# Autodesk Inventor assembly: Ensamblaje1
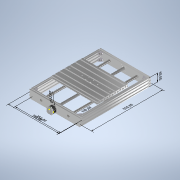
[picture p0: Inventor's stored thumbnail of the model, 180x180]
Saved by Autodesk Inventor 2021 (Build 250183000, 183)
## iProperties
Created: 2022-05-21
Part Number: Ensamblaje1
Document SubType Name: Assembly
Designer: 79449
Author: 79449
## Documents named in this file (27)
- C:\Users\79449\Documents\CNC_DISENO_DE MAQUINAS\Piezas-Ensambles_Inventor\Primera_presentación\Ensamblaje1.iam
- C:\Users\79449\Documents\CNC_DISENO_DE MAQUINAS\Piezas-Ensambles_Inventor\Primera_presentación\V-SLOT_2060_26cm.ipt
- C:\Users\79449\Documents\CNC_DISENO_DE MAQUINAS\Piezas-Ensambles_Inventor\Primera_presentación\V-SLOT_2060_30cm.ipt
- C:\Users\79449\Documents\CNC_DISENO_DE MAQUINAS\Piezas-Ensambles_Inventor\Primera_presentación\SFU-1605.ipt
- C:\Users\79449\Documents\CNC_DISENO_DE MAQUINAS\Piezas-Ensambles_Inventor\Primera_presentación\Ball Screew.step.ipt
- C:\Users\79449\Documents\CNC_DISENO_DE MAQUINAS\Piezas-Ensambles_Inventor\Primera_presentación\EjeBase.ipt
- C:\Users\79449\Documents\CNC_DISENO_DE MAQUINAS\Piezas-Ensambles_Inventor\Primera_presentación\ball nut housing bracket holder.ipt
- C:\Users\79449\Documents\CNC_DISENO_DE MAQUINAS\Piezas-Ensambles_Inventor\Primera_presentación\Chumacera\chumacera de 20 mm.iam
- C:\Users\79449\Documents\CNC_DISENO_DE MAQUINAS\Piezas-Ensambles_Inventor\Primera_presentación\T_20240.ipt
- C:\Users\79449\Documents\Inventor\Content Center Files\R2021\es-ES\AS 1427(05)\AS 1427 - M8 x 30(5) II.ipt
- C:\Users\79449\Documents\CNC_DISENO_DE MAQUINAS\Piezas-Ensambles_Inventor\Primera_presentación\PiezaNivel.ipt
- C:\Users\79449\Documents\Inventor\Content Center Files\R2021\es-ES\AS 1427(05)\AS 1427 - M4 x 20(5) II.ipt
- C:\Users\79449\Documents\CNC_DISENO_DE MAQUINAS\Piezas-Ensambles_Inventor\Primera_presentación\Cast corner bracket-20x20x17.ipt
- C:\Users\79449\Documents\Inventor\Content Center Files\R2021\es-ES\ANSI_ASME B18.5\ANSI_ASME B18.5 - 1_4 - 20 - 7_16 - 1_4-20 UNC.ipt
- C:\Users\79449\Documents\CNC_DISENO_DE MAQUINAS\Piezas-Ensambles_Inventor\Primera_presentación\Cast corner bracket-20x20x17_MIR.ipt
- C:\Users\79449\Documents\CNC_DISENO_DE MAQUINAS\Piezas-Ensambles_Inventor\Primera_presentación\Cast corner bracket-20x20x17_MIR1.ipt
- C:\Users\79449\Documents\CNC_DISENO_DE MAQUINAS\Piezas-Ensambles_Inventor\Primera_presentación\Cast corner bracket-20x20x17_MIR_MIR.ipt
- C:\Users\79449\Documents\Inventor\Content Center Files\R2021\es-ES\ANSI B18.2.2(08)\ANSI B18.2.2 - 1_4 - 20(3).ipt
- C:\Users\79449\Documents\Inventor\Content Center Files\R2021\es-ES\SAE J773b\SAE J773b - 3_8. SAE Tipo L. Fino.ipt
- C:\Users\79449\Documents\Inventor\Content Center Files\R2021\es-ES\AS 1112 (2)\AS 1112 - M8  Tipo 10.ipt
- C:\Users\79449\Documents\CNC_DISENO_DE MAQUINAS\Piezas-Ensambles_Inventor\Primera_presentación\Cast corner bracket-20x20x17_MIR2.ipt
- C:\Users\79449\Documents\CNC_DISENO_DE MAQUINAS\Piezas-Ensambles_Inventor\Primera_presentación\Cast corner bracket-20x20x17_MIR_MIR1.ipt
- C:\Users\79449\Documents\CNC_DISENO_DE MAQUINAS\Piezas-Ensambles_Inventor\Primera_presentación\Cast corner bracket-20x20x17_MIR1_MIR.ipt
- C:\Users\79449\Documents\CNC_DISENO_DE MAQUINAS\Piezas-Ensambles_Inventor\Primera_presentación\Cast corner bracket-20x20x17_MIR_MIR_MIR.ipt
- C:\Users\79449\Documents\CNC_DISENO_DE MAQUINAS\Piezas-Ensambles_Inventor\Primera_presentación\Nema17\Assembly1.iam
- C:\Users\79449\Documents\CNC_DISENO_DE MAQUINAS\Piezas-Ensambles_Inventor\Primera_presentación\Flexible Coupling 16-5.ipt
- C:\Users\79449\Documents\Inventor\Content Center Files\R2021\es-ES\U 3284(2)\Unbrako. Hallowell Steel Collars. Inch Series - 0.625 x 1 1_8 x 1_2.ipt
## Components (72 placed, 27 different names)
1. V-SLOT_2060_51cm:1 — Coincidencia:1, Coincidencia:3, Coincidencia:4, Coincidencia:6, Coincidencia:10, Coincidencia:11, Coincidencia:12, Coincidencia:52, Coincidencia:63
2. V-SLOT_2060_30cm:1 — Coincidencia:8, Coincidencia:10, Coincidencia:12, Coincidencia:14, Coincidencia:17, Coincidencia:19, Coincidencia:53, Coincidencia:60, Simetría:1
3. V-SLOT_2060_51cm:2 — Coincidencia:2, Coincidencia:3, Coincidencia:13
4. V-SLOT_2060_39cm:2 — Coincidencia:4, Coincidencia:5, Coincidencia:6, Coincidencia:13, Coincidencia:18, Coincidencia:20, Nivelación:3, Simetría:1, Ángulo:2, Coincidencia:124, Coincidencia:125, Coincidencia:131
5. SFU-1605:1 — Coincidencia:16, Coincidencia:21, Nivelación:1, Coincidencia:22
6. Ball Screew.step:1 — Coincidencia:14, Coincidencia:16, Coincidencia:126, Coincidencia:129
7. EjeBase:1 — Coincidencia:17, Coincidencia:18, Coincidencia:24
8. EjeBase:2 — Coincidencia:19, Coincidencia:20, Coincidencia:23, Coincidencia:130
9. ball nut housing bracket holder:1 — Coincidencia:21, Nivelación:1, Coincidencia:22, Ángulo:1, Coincidencia:38, Coincidencia:39
10. chumacera de 20 mm:1 [sub-assembly] — Coincidencia:23, Coincidencia:25, Coincidencia:35, Coincidencia:87, Coincidencia:89
11. chumacera de 20 mm:2 [sub-assembly] — Coincidencia:24, Coincidencia:26, Coincidencia:29, Coincidencia:31, Coincidencia:91, Coincidencia:93
12. T_20240:1 — Coincidencia:25, Coincidencia:26, Coincidencia:27, Coincidencia:28, Coincidencia:30, Coincidencia:32, Coincidencia:33, Coincidencia:34, Coincidencia:35, Coincidencia:36, Coincidencia:37, Ángulo:1, Coincidencia:41, Coincidencia:43, Coincidencia:45, Coincidencia:46, Coincidencia:47, Coincidencia:48, Coincidencia:49, Coincidencia:50
13. AS 1427 H - Métrico M8 x 30:1 — Coincidencia:34, Coincidencia:37, Coincidencia:88, Coincidencia:100
14. AS 1427 H - Métrico M8 x 30:3 — Coincidencia:33, Coincidencia:36, Coincidencia:86, Coincidencia:98
15. AS 1427 H - Métrico M8 x 30:4 — Coincidencia:27, Coincidencia:28, Coincidencia:29, Coincidencia:92, Coincidencia:94
16. AS 1427 H - Métrico M8 x 30:7 — Coincidencia:30, Coincidencia:31, Coincidencia:32, Coincidencia:90, Coincidencia:96
17. PiezaNivel:1 — Coincidencia:38, Coincidencia:39, Coincidencia:51
18. AS 1427 H - Métrico M4 x 20:1 — Coincidencia:41, Coincidencia:49
19. AS 1427 H - Métrico M4 x 20:2 — Coincidencia:43, Coincidencia:46
20. AS 1427 H - Métrico M4 x 20:3 — Coincidencia:45, Coincidencia:50
21. AS 1427 H - Métrico M4 x 20:5 — Coincidencia:47, Coincidencia:48, Coincidencia:51
22. Cast corner bracket-20x20x17:2 — Coincidencia:52, Coincidencia:53, Coincidencia:61, Coincidencia:62, Coincidencia:64, Coincidencia:71, Coincidencia:73
23. Perno de cabeza en T - Pulgadas 1/4 - 20 - 7/16:1 — Coincidencia:60, Coincidencia:61, Coincidencia:72
24. Perno de cabeza en T - Pulgadas 1/4 - 20 - 7/16:2 — Coincidencia:62, Coincidencia:63, Coincidencia:70
25. Cast corner bracket-20x20x17_MIR:1 — Coincidencia:65, Coincidencia:75, Coincidencia:77
26. Perno de cabeza en T - Pulgadas 1/4 - 20 - 7/16:3 — Coincidencia:76
27. Perno de cabeza en T - Pulgadas 1/4 - 20 - 7/16:4 — Coincidencia:74
28. Cast corner bracket-20x20x17_MIR1:1 — Coincidencia:66, Coincidencia:83, Coincidencia:85
29. Perno de cabeza en T - Pulgadas 1/4 - 20 - 7/16:5 — Coincidencia:84
30. Perno de cabeza en T - Pulgadas 1/4 - 20 - 7/16:6 — Coincidencia:82
31. Cast corner bracket-20x20x17_MIR_MIR:1 — Coincidencia:69, Coincidencia:79, Coincidencia:81
32. Perno de cabeza en T - Pulgadas 1/4 - 20 - 7/16:7 — Coincidencia:78
33. Perno de cabeza en T - Pulgadas 1/4 - 20 - 7/16:8 — Coincidencia:80
34. Tuerca de apriete hex - Pulgadas 1/4 - 20:1 — Coincidencia:70, Coincidencia:71
35. Tuerca de apriete hex - Pulgadas 1/4 - 20:2 — Coincidencia:72, Coincidencia:73
36. Tuerca de apriete hex - Pulgadas 1/4 - 20:3 — Coincidencia:74, Coincidencia:75
37. Tuerca de apriete hex - Pulgadas 1/4 - 20:4 — Coincidencia:76, Coincidencia:77
38. Tuerca de apriete hex - Pulgadas 1/4 - 20:5 — Coincidencia:78, Coincidencia:79
39. Tuerca de apriete hex - Pulgadas 1/4 - 20:6 — Coincidencia:80, Coincidencia:81
40. Tuerca de apriete hex - Pulgadas 1/4 - 20:7 — Coincidencia:82, Coincidencia:83
41. Tuerca de apriete hex - Pulgadas 1/4 - 20:8 — Coincidencia:84, Coincidencia:85
42. Arandela elástica SAE J773b (Pulgadas) 3/8. SAE Tipo L. Fino:1 — Coincidencia:86, Coincidencia:87, Coincidencia:99
43. Arandela elástica SAE J773b (Pulgadas) 3/8. SAE Tipo L. Fino:2 — Coincidencia:88, Coincidencia:89, Coincidencia:101
44. Arandela elástica SAE J773b (Pulgadas) 3/8. SAE Tipo L. Fino:3 — Coincidencia:90, Coincidencia:91, Coincidencia:97
45. Arandela elástica SAE J773b (Pulgadas) 3/8. SAE Tipo L. Fino:4 — Coincidencia:92, Coincidencia:93, Coincidencia:95
46. AS 1112 (2) - Métrico M8  Tipo 10:1 — Coincidencia:94, Coincidencia:95
47. AS 1112 (2) - Métrico M8  Tipo 10:2 — Coincidencia:96, Coincidencia:97
48. AS 1112 (2) - Métrico M8  Tipo 10:3 — Coincidencia:98, Coincidencia:99
49. AS 1112 (2) - Métrico M8  Tipo 10:4 — Coincidencia:100, Coincidencia:101
50. Cast corner bracket-20x20x17_MIR2:1 — Coincidencia:102, Coincidencia:108, Coincidencia:110
51. Perno de cabeza en T - Pulgadas 1/4 - 20 - 7/16:9 — Coincidencia:111
52. Perno de cabeza en T - Pulgadas 1/4 - 20 - 7/16:10 — Coincidencia:109
53. Cast corner bracket-20x20x17_MIR_MIR1:1 — Coincidencia:105, Coincidencia:112, Coincidencia:114
54. Perno de cabeza en T - Pulgadas 1/4 - 20 - 7/16:11 — Coincidencia:115
55. Perno de cabeza en T - Pulgadas 1/4 - 20 - 7/16:12 — Coincidencia:113
56. Cast corner bracket-20x20x17_MIR1_MIR:1 — Coincidencia:106, Coincidencia:120, Coincidencia:122
57. Perno de cabeza en T - Pulgadas 1/4 - 20 - 7/16:13 — Coincidencia:123
58. Perno de cabeza en T - Pulgadas 1/4 - 20 - 7/16:14 — Coincidencia:121
59. Cast corner bracket-20x20x17_MIR_MIR_MIR:1 — Coincidencia:107, Coincidencia:116, Coincidencia:118
60. Perno de cabeza en T - Pulgadas 1/4 - 20 - 7/16:15 — Coincidencia:117
61. Perno de cabeza en T - Pulgadas 1/4 - 20 - 7/16:16 — Coincidencia:119
62. Tuerca de apriete hex - Pulgadas 1/4 - 20:9 — Coincidencia:108, Coincidencia:109
63. Tuerca de apriete hex - Pulgadas 1/4 - 20:10 — Coincidencia:110, Coincidencia:111
64. Tuerca de apriete hex - Pulgadas 1/4 - 20:11 — Coincidencia:112, Coincidencia:113
65. Tuerca de apriete hex - Pulgadas 1/4 - 20:12 — Coincidencia:114, Coincidencia:115
66. Tuerca de apriete hex - Pulgadas 1/4 - 20:13 — Coincidencia:116, Coincidencia:117
67. Tuerca de apriete hex - Pulgadas 1/4 - 20:14 — Coincidencia:118, Coincidencia:119
68. Tuerca de apriete hex - Pulgadas 1/4 - 20:15 — Coincidencia:120, Coincidencia:121
69. Tuerca de apriete hex - Pulgadas 1/4 - 20:16 — Coincidencia:122, Coincidencia:123
70. Assembly1:1 [sub-assembly] — Ángulo:2, Coincidencia:124, Coincidencia:125, Coincidencia:127, Coincidencia:128
71. Flexible Coupling 16-5:1 — Coincidencia:126, Coincidencia:127, Coincidencia:128, Coincidencia:129
72. Anillo de ajuste 0.625 x 1 1/8 x 1/2:1 — Coincidencia:130, Coincidencia:131
## Relationships (121: Mate 115, Flush 3, Angle 2, Symmetry 1)
- Coincidencia:1 [Mate]: V-SLOT_2060_51cm:1
- Coincidencia:2 [Mate]: V-SLOT_2060_51cm:2
- Coincidencia:3 [Mate] (350 mm): V-SLOT_2060_51cm:1 ↔ V-SLOT_2060_51cm:2
- Coincidencia:4 [Mate]: V-SLOT_2060_51cm:1 ↔ V-SLOT_2060_39cm:2
- Coincidencia:5 [Mate]: V-SLOT_2060_39cm:2
- Coincidencia:6 [Mate]: V-SLOT_2060_51cm:1 ↔ V-SLOT_2060_39cm:2
- Coincidencia:8 [Mate]: V-SLOT_2060_30cm:1
- Coincidencia:10 [Mate]: V-SLOT_2060_51cm:1 ↔ V-SLOT_2060_30cm:1
- Coincidencia:11 [Mate]: V-SLOT_2060_51cm:1
- Coincidencia:12 [Mate]: V-SLOT_2060_51cm:1 ↔ V-SLOT_2060_30cm:1
- Coincidencia:13 [Mate]: V-SLOT_2060_51cm:2 ↔ V-SLOT_2060_39cm:2
- Coincidencia:14 [Mate]: V-SLOT_2060_30cm:1 ↔ Ball Screew.step:1
- Coincidencia:16 [Mate]: SFU-1605:1 ↔ Ball Screew.step:1
- Coincidencia:17 [Mate]: V-SLOT_2060_30cm:1 ↔ EjeBase:1
- Coincidencia:18 [Mate]: V-SLOT_2060_39cm:2 ↔ EjeBase:1
- Coincidencia:19 [Mate]: V-SLOT_2060_30cm:1 ↔ EjeBase:2
- Coincidencia:20 [Mate]: V-SLOT_2060_39cm:2 ↔ EjeBase:2
- Coincidencia:21 [Mate]: SFU-1605:1 ↔ ball nut housing bracket holder:1
- Nivelación:1 [Flush]: SFU-1605:1 ↔ ball nut housing bracket holder:1
- Coincidencia:22 [Mate]: SFU-1605:1 ↔ ball nut housing bracket holder:1
- Coincidencia:23 [Mate]: EjeBase:2 ↔ chumacera de 20 mm:1
- Coincidencia:24 [Mate]: EjeBase:1 ↔ chumacera de 20 mm:2
- Coincidencia:25 [Mate]: chumacera de 20 mm:1 ↔ T_20240:1
- Coincidencia:26 [Mate]: chumacera de 20 mm:2 ↔ T_20240:1
- Coincidencia:27 [Mate]: T_20240:1 ↔ AS 1427 H - Métrico M8 x 30:4
- Coincidencia:28 [Mate]: T_20240:1 ↔ AS 1427 H - Métrico M8 x 30:4
- Coincidencia:29 [Mate]: chumacera de 20 mm:2 ↔ AS 1427 H - Métrico M8 x 30:4
- Coincidencia:30 [Mate]: T_20240:1 ↔ AS 1427 H - Métrico M8 x 30:7
- Coincidencia:31 [Mate]: chumacera de 20 mm:2 ↔ AS 1427 H - Métrico M8 x 30:7
- Coincidencia:32 [Mate]: T_20240:1 ↔ AS 1427 H - Métrico M8 x 30:7
- Coincidencia:33 [Mate]: T_20240:1 ↔ AS 1427 H - Métrico M8 x 30:3
- Coincidencia:34 [Mate]: T_20240:1 ↔ AS 1427 H - Métrico M8 x 30:1
- Coincidencia:35 [Mate] (7 mm): chumacera de 20 mm:1 ↔ T_20240:1
- Coincidencia:36 [Mate]: T_20240:1 ↔ AS 1427 H - Métrico M8 x 30:3
- Coincidencia:37 [Mate]: T_20240:1 ↔ AS 1427 H - Métrico M8 x 30:1
- Ángulo:1 [Angle] (-180 deg): ball nut housing bracket holder:1 ↔ T_20240:1
- Coincidencia:38 [Mate]: ball nut housing bracket holder:1 ↔ PiezaNivel:1
- Coincidencia:39 [Mate]: ball nut housing bracket holder:1 ↔ PiezaNivel:1
- Coincidencia:41 [Mate]: T_20240:1 ↔ AS 1427 H - Métrico M4 x 20:1
- Coincidencia:43 [Mate]: T_20240:1 ↔ AS 1427 H - Métrico M4 x 20:2
- Coincidencia:45 [Mate]: T_20240:1 ↔ AS 1427 H - Métrico M4 x 20:3
- Coincidencia:46 [Mate]: T_20240:1 ↔ AS 1427 H - Métrico M4 x 20:2
- Coincidencia:47 [Mate]: T_20240:1 ↔ AS 1427 H - Métrico M4 x 20:5
- Coincidencia:48 [Mate]: T_20240:1 ↔ AS 1427 H - Métrico M4 x 20:5
- Coincidencia:49 [Mate]: T_20240:1 ↔ AS 1427 H - Métrico M4 x 20:1
- Coincidencia:50 [Mate]: T_20240:1 ↔ AS 1427 H - Métrico M4 x 20:3
- Coincidencia:51 [Mate]: PiezaNivel:1 ↔ AS 1427 H - Métrico M4 x 20:5
- Coincidencia:52 [Mate]: V-SLOT_2060_51cm:1 ↔ Cast corner bracket-20x20x17:2
- Coincidencia:53 [Mate]: V-SLOT_2060_30cm:1 ↔ Cast corner bracket-20x20x17:2
- Coincidencia:60 [Mate]: V-SLOT_2060_30cm:1 ↔ Perno de cabeza en T - Pulgadas 1/4 - 20 - 7/16:1
- Coincidencia:61 [Mate]: Cast corner bracket-20x20x17:2 ↔ Perno de cabeza en T - Pulgadas 1/4 - 20 - 7/16:1
- Coincidencia:62 [Mate]: Cast corner bracket-20x20x17:2 ↔ Perno de cabeza en T - Pulgadas 1/4 - 20 - 7/16:2
- Coincidencia:63 [Mate]: V-SLOT_2060_51cm:1 ↔ Perno de cabeza en T - Pulgadas 1/4 - 20 - 7/16:2
- Coincidencia:64 [Mate]: Cast corner bracket-20x20x17:2
- Nivelación:2 [Flush] (195 mm)
- Coincidencia:65 [Mate]: Cast corner bracket-20x20x17_MIR:1
- Nivelación:3 [Flush] (-275 mm): V-SLOT_2060_39cm:2
- Coincidencia:66 [Mate]: Cast corner bracket-20x20x17_MIR1:1
- Coincidencia:69 [Mate]: Cast corner bracket-20x20x17_MIR_MIR:1
- Coincidencia:70 [Mate]: Perno de cabeza en T - Pulgadas 1/4 - 20 - 7/16:2 ↔ Tuerca de apriete hex - Pulgadas 1/4 - 20:1
- Coincidencia:71 [Mate]: Cast corner bracket-20x20x17:2 ↔ Tuerca de apriete hex - Pulgadas 1/4 - 20:1
- Coincidencia:72 [Mate]: Perno de cabeza en T - Pulgadas 1/4 - 20 - 7/16:1 ↔ Tuerca de apriete hex - Pulgadas 1/4 - 20:2
- Coincidencia:73 [Mate]: Cast corner bracket-20x20x17:2 ↔ Tuerca de apriete hex - Pulgadas 1/4 - 20:2
- Coincidencia:74 [Mate]: Perno de cabeza en T - Pulgadas 1/4 - 20 - 7/16:4 ↔ Tuerca de apriete hex - Pulgadas 1/4 - 20:3
- Coincidencia:75 [Mate]: Cast corner bracket-20x20x17_MIR:1 ↔ Tuerca de apriete hex - Pulgadas 1/4 - 20:3
- Coincidencia:76 [Mate]: Perno de cabeza en T - Pulgadas 1/4 - 20 - 7/16:3 ↔ Tuerca de apriete hex - Pulgadas 1/4 - 20:4
- Coincidencia:77 [Mate]: Cast corner bracket-20x20x17_MIR:1 ↔ Tuerca de apriete hex - Pulgadas 1/4 - 20:4
- Coincidencia:78 [Mate]: Perno de cabeza en T - Pulgadas 1/4 - 20 - 7/16:7 ↔ Tuerca de apriete hex - Pulgadas 1/4 - 20:5
- Coincidencia:79 [Mate]: Cast corner bracket-20x20x17_MIR_MIR:1 ↔ Tuerca de apriete hex - Pulgadas 1/4 - 20:5
- Coincidencia:80 [Mate]: Perno de cabeza en T - Pulgadas 1/4 - 20 - 7/16:8 ↔ Tuerca de apriete hex - Pulgadas 1/4 - 20:6
- Coincidencia:81 [Mate]: Cast corner bracket-20x20x17_MIR_MIR:1 ↔ Tuerca de apriete hex - Pulgadas 1/4 - 20:6
- Coincidencia:82 [Mate]: Perno de cabeza en T - Pulgadas 1/4 - 20 - 7/16:6 ↔ Tuerca de apriete hex - Pulgadas 1/4 - 20:7
- Coincidencia:83 [Mate]: Cast corner bracket-20x20x17_MIR1:1 ↔ Tuerca de apriete hex - Pulgadas 1/4 - 20:7
- Coincidencia:84 [Mate]: Perno de cabeza en T - Pulgadas 1/4 - 20 - 7/16:5 ↔ Tuerca de apriete hex - Pulgadas 1/4 - 20:8
- Coincidencia:85 [Mate]: Cast corner bracket-20x20x17_MIR1:1 ↔ Tuerca de apriete hex - Pulgadas 1/4 - 20:8
- Coincidencia:86 [Mate]: AS 1427 H - Métrico M8 x 30:3 ↔ Arandela elástica SAE J773b (Pulgadas) 3/8. SAE Tipo L. Fino:1
- Coincidencia:87 [Mate]: chumacera de 20 mm:1 ↔ Arandela elástica SAE J773b (Pulgadas) 3/8. SAE Tipo L. Fino:1
- Coincidencia:88 [Mate]: AS 1427 H - Métrico M8 x 30:1 ↔ Arandela elástica SAE J773b (Pulgadas) 3/8. SAE Tipo L. Fino:2
- Coincidencia:89 [Mate]: chumacera de 20 mm:1 ↔ Arandela elástica SAE J773b (Pulgadas) 3/8. SAE Tipo L. Fino:2
- Coincidencia:90 [Mate]: AS 1427 H - Métrico M8 x 30:7 ↔ Arandela elástica SAE J773b (Pulgadas) 3/8. SAE Tipo L. Fino:3
- Coincidencia:91 [Mate]: chumacera de 20 mm:2 ↔ Arandela elástica SAE J773b (Pulgadas) 3/8. SAE Tipo L. Fino:3
- Coincidencia:92 [Mate]: AS 1427 H - Métrico M8 x 30:4 ↔ Arandela elástica SAE J773b (Pulgadas) 3/8. SAE Tipo L. Fino:4
- Coincidencia:93 [Mate]: chumacera de 20 mm:2 ↔ Arandela elástica SAE J773b (Pulgadas) 3/8. SAE Tipo L. Fino:4
- Coincidencia:94 [Mate]: AS 1427 H - Métrico M8 x 30:4 ↔ AS 1112 (2) - Métrico M8  Tipo 10:1
- Coincidencia:95 [Mate]: Arandela elástica SAE J773b (Pulgadas) 3/8. SAE Tipo L. Fino:4 ↔ AS 1112 (2) - Métrico M8  Tipo 10:1
- Coincidencia:96 [Mate]: AS 1427 H - Métrico M8 x 30:7 ↔ AS 1112 (2) - Métrico M8  Tipo 10:2
- Coincidencia:97 [Mate]: Arandela elástica SAE J773b (Pulgadas) 3/8. SAE Tipo L. Fino:3 ↔ AS 1112 (2) - Métrico M8  Tipo 10:2
- Coincidencia:98 [Mate]: AS 1427 H - Métrico M8 x 30:3 ↔ AS 1112 (2) - Métrico M8  Tipo 10:3
- Coincidencia:99 [Mate]: Arandela elástica SAE J773b (Pulgadas) 3/8. SAE Tipo L. Fino:1 ↔ AS 1112 (2) - Métrico M8  Tipo 10:3
- Coincidencia:100 [Mate]: AS 1427 H - Métrico M8 x 30:1 ↔ AS 1112 (2) - Métrico M8  Tipo 10:4
- Coincidencia:101 [Mate]: Arandela elástica SAE J773b (Pulgadas) 3/8. SAE Tipo L. Fino:2 ↔ AS 1112 (2) - Métrico M8  Tipo 10:4
- Simetría:1 [Symmetry]: V-SLOT_2060_30cm:1 ↔ V-SLOT_2060_39cm:2
- Coincidencia:102 [Mate]: Cast corner bracket-20x20x17_MIR2:1
- Coincidencia:105 [Mate]: Cast corner bracket-20x20x17_MIR_MIR1:1
- Coincidencia:106 [Mate]: Cast corner bracket-20x20x17_MIR1_MIR:1
- Coincidencia:107 [Mate]: Cast corner bracket-20x20x17_MIR_MIR_MIR:1
- Coincidencia:108 [Mate]: Cast corner bracket-20x20x17_MIR2:1 ↔ Tuerca de apriete hex - Pulgadas 1/4 - 20:9
- Coincidencia:109 [Mate]: Perno de cabeza en T - Pulgadas 1/4 - 20 - 7/16:10 ↔ Tuerca de apriete hex - Pulgadas 1/4 - 20:9
- Coincidencia:110 [Mate]: Cast corner bracket-20x20x17_MIR2:1 ↔ Tuerca de apriete hex - Pulgadas 1/4 - 20:10
- Coincidencia:111 [Mate]: Perno de cabeza en T - Pulgadas 1/4 - 20 - 7/16:9 ↔ Tuerca de apriete hex - Pulgadas 1/4 - 20:10
- Coincidencia:112 [Mate]: Cast corner bracket-20x20x17_MIR_MIR1:1 ↔ Tuerca de apriete hex - Pulgadas 1/4 - 20:11
- Coincidencia:113 [Mate]: Perno de cabeza en T - Pulgadas 1/4 - 20 - 7/16:12 ↔ Tuerca de apriete hex - Pulgadas 1/4 - 20:11
- Coincidencia:114 [Mate]: Cast corner bracket-20x20x17_MIR_MIR1:1 ↔ Tuerca de apriete hex - Pulgadas 1/4 - 20:12
- Coincidencia:115 [Mate]: Perno de cabeza en T - Pulgadas 1/4 - 20 - 7/16:11 ↔ Tuerca de apriete hex - Pulgadas 1/4 - 20:12
- Coincidencia:116 [Mate]: Cast corner bracket-20x20x17_MIR_MIR_MIR:1 ↔ Tuerca de apriete hex - Pulgadas 1/4 - 20:13
- Coincidencia:117 [Mate]: Perno de cabeza en T - Pulgadas 1/4 - 20 - 7/16:15 ↔ Tuerca de apriete hex - Pulgadas 1/4 - 20:13
- Coincidencia:118 [Mate]: Cast corner bracket-20x20x17_MIR_MIR_MIR:1 ↔ Tuerca de apriete hex - Pulgadas 1/4 - 20:14
- Coincidencia:119 [Mate]: Perno de cabeza en T - Pulgadas 1/4 - 20 - 7/16:16 ↔ Tuerca de apriete hex - Pulgadas 1/4 - 20:14
- Coincidencia:120 [Mate]: Cast corner bracket-20x20x17_MIR1_MIR:1 ↔ Tuerca de apriete hex - Pulgadas 1/4 - 20:15
- Coincidencia:121 [Mate]: Perno de cabeza en T - Pulgadas 1/4 - 20 - 7/16:14 ↔ Tuerca de apriete hex - Pulgadas 1/4 - 20:15
- Coincidencia:122 [Mate]: Cast corner bracket-20x20x17_MIR1_MIR:1 ↔ Tuerca de apriete hex - Pulgadas 1/4 - 20:16
- Coincidencia:123 [Mate]: Perno de cabeza en T - Pulgadas 1/4 - 20 - 7/16:13 ↔ Tuerca de apriete hex - Pulgadas 1/4 - 20:16
- Ángulo:2 [Angle] (0 deg): V-SLOT_2060_39cm:2 ↔ Assembly1:1
- Coincidencia:124 [Mate]: V-SLOT_2060_39cm:2 ↔ Assembly1:1
- Coincidencia:125 [Mate]: V-SLOT_2060_39cm:2 ↔ Assembly1:1
- Coincidencia:126 [Mate]: Ball Screew.step:1 ↔ Flexible Coupling 16-5:1
- Coincidencia:127 [Mate]: Assembly1:1 ↔ Flexible Coupling 16-5:1
- Coincidencia:128 [Mate]: Assembly1:1 ↔ Flexible Coupling 16-5:1
- Coincidencia:129 [Mate]: Ball Screew.step:1 ↔ Flexible Coupling 16-5:1
- Coincidencia:130 [Mate]: EjeBase:2 ↔ Anillo de ajuste 0.625 x 1 1/8 x 1/2:1
- Coincidencia:131 [Mate]: V-SLOT_2060_39cm:2 ↔ Anillo de ajuste 0.625 x 1 1/8 x 1/2:1
